# Autodesk Inventor assembly: Flywheels
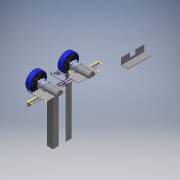
[picture p0: Inventor's stored thumbnail of the model, 180x180]
Saved by Autodesk Inventor 2017 (Build 210142000, 142)
## iProperties
Created: 2016-10-19
Part Number: Flywheels
Document SubType Name: Assembly
Designer: Aditya
Author: Aditya
## Documents named in this file (9)
- C:\Users\Aditya\Documents\GitHub\RobotuxCAD\Team Robotux 15-16 Robot Cad Assets\Flywheels.iam
- C:\Users\Aditya\Documents\GitHub\RobotuxCAD\Team Robotux 15-16 Robot Cad Assets\Flywheel w motor.iam
- C:\Users\Aditya\Documents\GitHub\RobotuxCAD\Team Robotux 15-16 Robot Cad Assets\flywheel plate.ipt
- C:\Users\Aditya\Documents\GitHub\RobotuxCAD\Team Robotux 15-16 Robot Cad Assets\Flywheel Headpiece.ipt
- C:\Users\Aditya\Documents\GitHub\RobotuxCAD\Team Robotux 15-16 Robot Cad Assets\Flywheel w motor_MIR.iam
- C:\Users\Aditya\Documents\GitHub\RobotuxCAD\Team Robotux 15-16 Robot Cad Assets\flywheel plate_MIR.ipt
- C:\Users\Aditya\Documents\GitHub\RobotuxCAD\Team Robotux 15-16 Robot Cad Assets\Long Boi.ipt
- C:\Users\Aditya\Documents\GitHub\RobotuxCAD\Team Robotux 15-16 Robot Cad Assets\Long Boi_MIR.ipt
- C:\Users\Aditya\Documents\GitHub\RobotuxCAD\Team Robotux 15-16 Robot Cad Assets\cut top wheel mout thingy.ipt
## Components (8 placed, 8 different names)
1. Flywheel w motor:1 [sub-assembly] — Mate:1, Flush:1, Mate:2
2. flywheel plate:1 — Mate:1, Flush:1, Mate:2, Mate:5, Mate:7, Mate:8, Mate:11, Mate:12, Mate:16
3. Flywheel Headpiece:1 — Mate:5, Mate:6, Mate:7, Mate:8, Mate:9, Mate:10, Mate:11, Mate:12, Mate:13, Mate:14, Mate:15, Flush:3, Mate:17, Flush:4
4. Flywheel w motor_MIR:1 [sub-assembly] — Mate:3, Flush:2, Mate:4
5. flywheel plate_MIR:1 — Mate:3, Flush:2, Mate:4, Mate:6, Mate:9, Mate:10, Mate:13, Mate:14, Mate:18
6. Long Boi:1 — Mate:17, Flush:4, Mate:18
7. Long Boi_MIR:1 — Mate:15, Flush:3, Mate:16
8. cut top wheel mout thingy:1
## Relationships (22: Mate 18, Flush 4)
- Mate:1: Flywheel w motor:1 ↔ flywheel plate:1
- Flush:1: Flywheel w motor:1 ↔ flywheel plate:1
- Mate:2: Flywheel w motor:1 ↔ flywheel plate:1
- Mate:3: Flywheel w motor_MIR:1 ↔ flywheel plate_MIR:1
- Flush:2: Flywheel w motor_MIR:1 ↔ flywheel plate_MIR:1
- Mate:4: Flywheel w motor_MIR:1 ↔ flywheel plate_MIR:1
- Mate:5: flywheel plate:1 ↔ Flywheel Headpiece:1
- Mate:6: Flywheel Headpiece:1 ↔ flywheel plate_MIR:1
- Mate:7: flywheel plate:1 ↔ Flywheel Headpiece:1
- Mate:8: flywheel plate:1 ↔ Flywheel Headpiece:1
- Mate:9: Flywheel Headpiece:1 ↔ flywheel plate_MIR:1
- Mate:10: Flywheel Headpiece:1 ↔ flywheel plate_MIR:1
- Mate:11: flywheel plate:1 ↔ Flywheel Headpiece:1
- Mate:12: flywheel plate:1 ↔ Flywheel Headpiece:1
- Mate:13: Flywheel Headpiece:1 ↔ flywheel plate_MIR:1
- Mate:14: Flywheel Headpiece:1 ↔ flywheel plate_MIR:1
- Mate:15: Flywheel Headpiece:1 ↔ Long Boi_MIR:1
- Flush:3: Flywheel Headpiece:1 ↔ Long Boi_MIR:1
- Mate:16: flywheel plate:1 ↔ Long Boi_MIR:1
- Mate:17: Flywheel Headpiece:1 ↔ Long Boi:1
- Flush:4: Flywheel Headpiece:1 ↔ Long Boi:1
- Mate:18: flywheel plate_MIR:1 ↔ Long Boi:1
